# Autodesk Inventor assembly: Shooter Curve Assembly
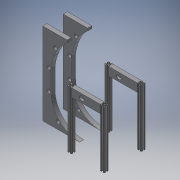
[picture p0: Inventor's stored thumbnail of the model, 180x180]
Saved by Autodesk Inventor 2018 (Build 220112000, 112)
## iProperties
Created: 2020-02-01
Part Number: Shooter Curve Assembly
Document SubType Name: Assembly
Designer: Weeb No1
Author: Weeb No1
## Documents named in this file (4)
- C:\Users\Weeb No1\Documents\GitHub\2020CAD\Gabriel Inventor Files (Shooter, Drivebase)\Shooter Curve Assembly\Main Assembly File\Shooter Curve Assembly.iam
- C:\Users\Weeb No1\Documents\GitHub\2020CAD\Gabriel Inventor Files (Shooter, Drivebase)\Shooter Curve Assembly\Part Files\Shooter Main Curve.ipt
- C:\Users\Weeb No1\Documents\GitHub\2020CAD\Gabriel Inventor Files (Shooter, Drivebase)\Shooter Curve Assembly\Part Files\8020 1010 x 14.ipt
- C:\Users\Weeb No1\Documents\GitHub\2020CAD\Gabriel Inventor Files (Shooter, Drivebase)\Shooter Curve Assembly\Part Files\1x2 5 in Beam Flywheel Mount.ipt
## Components (8 placed, 3 different names)
1. Shooter Main Curve:1 — Flush:1, Mate:1, Mate:2, Flush:2, Flush:3, Flush:18, Flush:20
2. 8020 1010 x 14:1 — Flush:1, Mate:1, Flush:5, Flush:6, Mate:7, Flush:11, Flush:14, Flush:18, Flush:23, Flush:24
3. 8020 1010 x 14:2 — Flush:4, Mate:3, Flush:7, Mate:9, Flush:15, Flush:19, Flush:22, Flush:25
4. Shooter Main Curve:2 — Mate:2, Flush:2, Flush:3, Flush:4, Mate:3, Flush:19, Flush:21
5. 8020 1010 x 14:3 — Flush:5, Flush:6, Flush:10, Flush:12, Flush:13, Flush:20, Mate:11, Flush:23
6. 8020 1010 x 14:4 — Flush:7, Flush:10, Flush:17, Flush:21, Mate:10, Flush:22
7. 1x2 5 in Beam Flywheel Mount:1 — Mate:9, Flush:15, Flush:17, Mate:10, Flush:25
8. 1x2 5 in Beam Flywheel Mount:2 — Mate:7, Flush:11, Flush:12, Flush:13, Flush:14, Mate:11, Flush:24
## Relationships (29: Flush 22, Mate 7)
- Flush:1 (203.2 mm): Shooter Main Curve:1 ↔ 8020 1010 x 14:1
- Mate:1 (25.4 mm): Shooter Main Curve:1 ↔ 8020 1010 x 14:1
- Mate:2 (101.6 mm): Shooter Main Curve:1 ↔ Shooter Main Curve:2
- Flush:2: Shooter Main Curve:1 ↔ Shooter Main Curve:2
- Flush:3: Shooter Main Curve:1 ↔ Shooter Main Curve:2
- Flush:4 (203.2 mm): 8020 1010 x 14:2 ↔ Shooter Main Curve:2
- Mate:3 (25.4 mm): 8020 1010 x 14:2 ↔ Shooter Main Curve:2
- Flush:5: 8020 1010 x 14:1 ↔ 8020 1010 x 14:3
- Flush:6: 8020 1010 x 14:1 ↔ 8020 1010 x 14:3
- Flush:7: 8020 1010 x 14:2 ↔ 8020 1010 x 14:4
- Flush:10: 8020 1010 x 14:3 ↔ 8020 1010 x 14:4
- Mate:7: 8020 1010 x 14:1 ↔ 1x2 5 in Beam Flywheel Mount:2
- Flush:11: 8020 1010 x 14:1 ↔ 1x2 5 in Beam Flywheel Mount:2
- Flush:12: 8020 1010 x 14:3 ↔ 1x2 5 in Beam Flywheel Mount:2
- Flush:13: 8020 1010 x 14:3 ↔ 1x2 5 in Beam Flywheel Mount:2
- Flush:14: 8020 1010 x 14:1 ↔ 1x2 5 in Beam Flywheel Mount:2
- Mate:9: 8020 1010 x 14:2 ↔ 1x2 5 in Beam Flywheel Mount:1
- Flush:15: 8020 1010 x 14:2 ↔ 1x2 5 in Beam Flywheel Mount:1
- Flush:17: 8020 1010 x 14:4 ↔ 1x2 5 in Beam Flywheel Mount:1
- Flush:18 (-38.1 mm): Shooter Main Curve:1 ↔ 8020 1010 x 14:1
- Flush:19 (-38.1 mm): 8020 1010 x 14:2 ↔ Shooter Main Curve:2
- Flush:20 (-38.1 mm): Shooter Main Curve:1 ↔ 8020 1010 x 14:3
- Flush:21 (-38.1 mm): Shooter Main Curve:2 ↔ 8020 1010 x 14:4
- Mate:10: 8020 1010 x 14:4 ↔ 1x2 5 in Beam Flywheel Mount:1
- Mate:11: 8020 1010 x 14:3 ↔ 1x2 5 in Beam Flywheel Mount:2
- Flush:22: 8020 1010 x 14:2 ↔ 8020 1010 x 14:4
- Flush:23: 8020 1010 x 14:1 ↔ 8020 1010 x 14:3
- Flush:24: 8020 1010 x 14:1 ↔ 1x2 5 in Beam Flywheel Mount:2
- Flush:25: 8020 1010 x 14:2 ↔ 1x2 5 in Beam Flywheel Mount:1
